# Autodesk Inventor assembly: gear
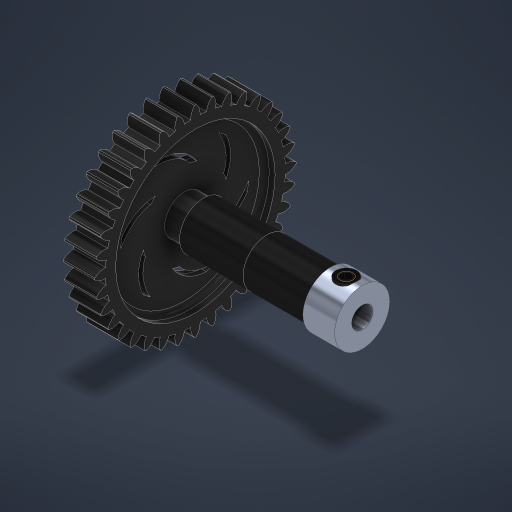
[picture p0: Inventor's stored thumbnail of the model, 512x512]
Saved by Autodesk Inventor 2024 (Build 280153000, 153)
## iProperties
Created: 2024-05-16
Part Number: gear
Document SubType Name: Assembly
Designer: avere
Author: avere
## Documents named in this file (8)
- C:\Users\avere\Documents\rbp_cad\kdot\chassis\drivebay\gear.iam
- C:\Users\avere\Documents\rbp_cad\VEX-CAD-Inventor-1.41\Motion\Gears\LS 36T Gear.ipt
- C:\Users\avere\Documents\rbp_cad\VEX-CAD-Inventor-1.41\Motion\Spacers\Spacer Nylon .375 OD\NSpacer .375 OD x .500.ipt
- C:\Users\avere\Documents\rbp_cad\VEX-CAD-Inventor-1.41\Motion\Spacers\Spacer Nylon .375 OD.ipt
- C:\Users\avere\Documents\rbp_cad\VEX-CAD-Inventor-1.41\Motion\Spacers\Washer Steel\SWasher .375 OD x .015625.ipt
- C:\Users\avere\Documents\rbp_cad\VEX-CAD-Inventor-1.41\Motion\Spacers\Washer Steel.ipt
- C:\Users\avere\Documents\rbp_cad\VEX-CAD-Inventor-1.41\Motion\Spacers\Washer Steel\SWasher .375 OD x .031250.ipt
- C:\Users\avere\Documents\rbp_cad\VEX-CAD-Inventor-1.41\Motion\Shaft LS\Shaft Collar ipts\Shaft Collar Set Screw.ipt
## Components (6 placed, 5 different names)
1. LS 36T Gear:1 — Insert:2, Insert:4
2. NSpacer .375 OD x .500:1 — Insert:3, Insert:4
3. NSpacer .375 OD x .500:2 — Insert:3, Insert:5
4. SWasher .375 OD x .015625:1 — Insert:1
5. SWasher .375 OD x .031250:2 — Insert:1, Insert:2
6. Shaft Collar Set Screw:1 — Insert:5
## Relationships (5: Insert 5)
- Insert:1: SWasher .375 OD x .015625:1 ↔ SWasher .375 OD x .031250:2
- Insert:2: LS 36T Gear:1 ↔ SWasher .375 OD x .031250:2
- Insert:3: NSpacer .375 OD x .500:1 ↔ NSpacer .375 OD x .500:2
- Insert:4: LS 36T Gear:1 ↔ NSpacer .375 OD x .500:1
- Insert:5: NSpacer .375 OD x .500:2 ↔ Shaft Collar Set Screw:1
